# Autodesk Inventor assembly: Assembly
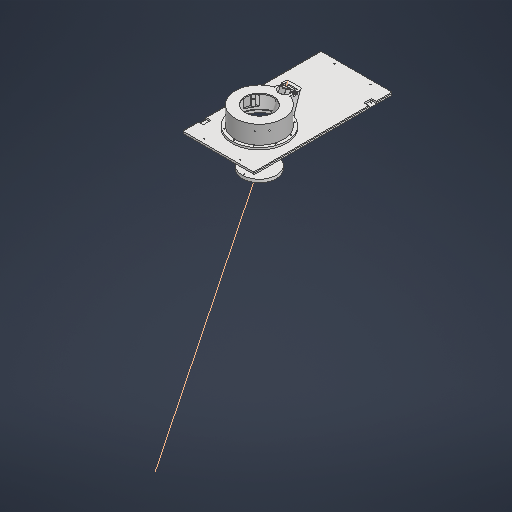
[picture p0: Inventor's stored thumbnail of the model, 512x512]
Saved by Autodesk Inventor 2026.1 (Build 301233000, 233)
## iProperties
Created: 2025-09-29
Part Number: Assembly
Document SubType Name: Assembly
Designer: mateo
Author: mateo
## Documents named in this file (5)
- C:\GitHub\In-situ-monitoring-of-powder-bed-fusion-additive-manufacturing\system_development\Mithril\v0.3\hardware_development\Assembly.iam
- C:\GitHub\In-situ-monitoring-of-powder-bed-fusion-additive-manufacturing\system_development\Mithril\v0.3\hardware_development\Cover Parts\Cylinder Housing Camera.ipt
- C:\GitHub\In-situ-monitoring-of-powder-bed-fusion-additive-manufacturing\system_development\Mithril\v0.3\hardware_development\Cover Parts\flircamera+lens.ipt
- C:\GitHub\In-situ-monitoring-of-powder-bed-fusion-additive-manufacturing\system_development\Mithril\v0.3\hardware_development\Cover Parts\substrate plate.ipt
- C:\GitHub\In-situ-monitoring-of-powder-bed-fusion-additive-manufacturing\system_development\Mithril\v0.3\hardware_development\Cover Parts\12mm Cover.ipt
## Components (4 placed, 4 different names)
1. Cylinder Housing Camera:1 — Insert:2, Insert:3, Insert:4
2. flircamera+lens:1 — Mate:1, Insert:3, Insert:4
3. substrate plate:1 — Rotational:1
4. 12mm Cover:1 — Insert:2, Rotational:1
## Relationships (5: Insert 3, Mate 1, RevoluteJoint 1)
- Mate:1: flircamera+lens:1
- Insert:2: Cylinder Housing Camera:1 ↔ 12mm Cover:1
- Rotational:1 [RevoluteJoint] (-150 mm): substrate plate:1 ↔ 12mm Cover:1
- Insert:3: Cylinder Housing Camera:1 ↔ flircamera+lens:1
- Insert:4: Cylinder Housing Camera:1 ↔ flircamera+lens:1
